# Autodesk Inventor assembly: SLBX
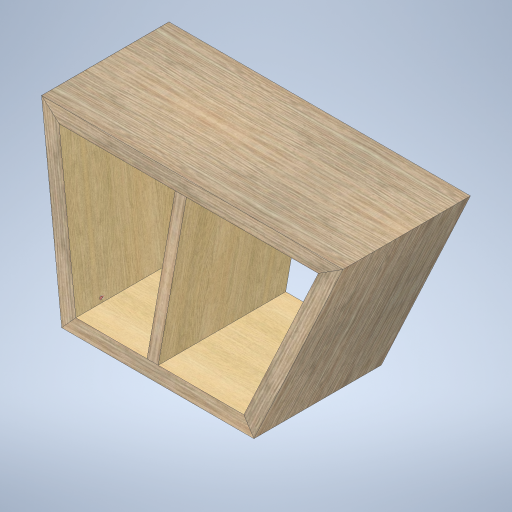
[picture p0: Inventor's stored thumbnail of the model, 512x512]
Saved by Autodesk Inventor 2024 (Build 280153000, 153)
## iProperties
Created: 2014-05-28
Part Number: SLBX
Document SubType Name: Assembly
Designer: SauliusD
Description: Slant Box
Author: SauliusD
## Documents named in this file (12)
- C:\W4INV 2024 Design\PROJECTS\Samples\Slant Box V3 Reception\Slant Box V2.iam
- C:\W4INV 2024 Design\PROJECTS\Samples\Slant Box V3 Reception\Top.ipt
- C:\W4INV 2024 Design\PROJECTS\Samples\Slant Box V3 Reception\Bottom.ipt
- C:\W4INV 2024 Design\PROJECTS\Samples\Slant Box V3 Reception\Left Side.ipt
- C:\W4INV 2024 Design\PROJECTS\Samples\Slant Box V3 Reception\Right Side.ipt
- C:\W4INV 2024 Design\PROJECTS\Samples\Slant Box V3 Reception\Partition.ipt
- C:\W4INV 2024 Design\PROJECTS\Samples\Slant Box V3 Reception\Slant Box V2.iam Smart Hardware\Clamex Joint11\Clamex Joint11.iam
- C:\W4INV 2024 Design\PROJECTS\Samples\Slant Box V3 Reception\Slant Box V2.iam Smart Hardware\Clamex Joint12\Clamex Joint12.iam
- C:\W4INV 2024 Design\PROJECTS\Samples\Slant Box V3 Reception\Slant Box V2.iam Smart Hardware\Clamex Joint13\Clamex Joint13.iam
- C:\W4INV 2024 Design\PROJECTS\Samples\Slant Box V3 Reception\Slant Box V2.iam Smart Hardware\Clamex Joint14\Clamex Joint14.iam
- C:\W4INV 2024 Design\PROJECTS\Samples\Slant Box V3 Reception\Slant Box V2.iam Smart Hardware\Clamex Joint15\Clamex Joint15.iam
- C:\W4INV 2024 Design\PROJECTS\Samples\Slant Box V3 Reception\Slant Box V2.iam Smart Hardware\Clamex Joint16\Clamex Joint16.iam
## Components (11 placed, 11 different names)
1. SLBX5;Right Side:1 — Flush:1, Flush:2, Flush:3
2. SLBX6;Top:1
3. SLBX2;Bottom:1
4. SLBX3;Left Side:1
5. SLBX4;Partition:1
6. Clamex Joint11:1 [sub-assembly]
7. Clamex Joint12:1 [sub-assembly]
8. Clamex Joint13:1 [sub-assembly]
9. Clamex Joint14:1 [sub-assembly]
10. Clamex Joint15:1 [sub-assembly]
11. Clamex Joint16:1 [sub-assembly]
## Relationships (3: Flush 3)
- Flush:1: SLBX5;Right Side:1
- Flush:2: SLBX5;Right Side:1
- Flush:3: SLBX5;Right Side:1
